# Autodesk Inventor assembly: Gripper Assembly
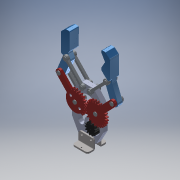
[picture p0: Inventor's stored thumbnail of the model, 180x180]
Saved by Autodesk Inventor 2019 (Build 230136000, 136)
## iProperties
Created: 2020-11-14
Part Number: Gripper Assembly
Document SubType Name: Assembly
Designer: micha
Author: micha
## Documents named in this file (12)
- D:\Files\ASU - Faculty of Engineering\Semester 10 - Spring 2021\Industrial Mechanisms and Robotics - MCT331\Four Bar Gripper Project\Gripper Assembly.iam
- D:\Files\ASU - Faculty of Engineering\Semester 10 - Spring 2021\Industrial Mechanisms and Robotics - MCT331\Four Bar Gripper Project\Part3_Base Gripper.ipt
- D:\Files\ASU - Faculty of Engineering\Semester 10 - Spring 2021\Industrial Mechanisms and Robotics - MCT331\Four Bar Gripper Project\Part4_Penggerak Kanan.ipt
- D:\Files\ASU - Faculty of Engineering\Semester 10 - Spring 2021\Industrial Mechanisms and Robotics - MCT331\Four Bar Gripper Project\Part5_Penggerak Kiri.ipt
- D:\Files\ASU - Faculty of Engineering\Semester 10 - Spring 2021\Industrial Mechanisms and Robotics - MCT331\Four Bar Gripper Project\Part1_Penjepit.ipt
- D:\Files\ASU - Faculty of Engineering\Semester 10 - Spring 2021\Industrial Mechanisms and Robotics - MCT331\Four Bar Gripper Project\Part2_Penyangga.ipt
- D:\Files\ASU - Faculty of Engineering\Semester 10 - Spring 2021\Industrial Mechanisms and Robotics - MCT331\Four Bar Gripper Project\Part6_Penyambung.ipt
- D:\Files\ASU - Faculty of Engineering\Semester 10 - Spring 2021\Industrial Mechanisms and Robotics - MCT331\Four Bar Gripper Project\Part7_Gripper to arm.ipt
- D:\Files\ASU - Faculty of Engineering\Semester 10 - Spring 2021\Industrial Mechanisms and Robotics - MCT331\Four Bar Gripper Project\Part8_to servo.ipt
- D:\Files\ASU - Faculty of Engineering\Semester 10 - Spring 2021\Industrial Mechanisms and Robotics - MCT331\Four Bar Gripper Project\Part1_Penjepit_V.ipt
- D:\Files\ASU - Faculty of Engineering\Semester 10 - Spring 2021\Industrial Mechanisms and Robotics - MCT331\Four Bar Gripper Project\Part1_Penjepit_Cutted.ipt
- D:\Files\ASU - Faculty of Engineering\Semester 10 - Spring 2021\Industrial Mechanisms and Robotics - MCT331\Four Bar Gripper Project\Part1_Penjepit_V_Cutted.ipt
## Components (29 placed, 10 different names)
1. Part3_Base Gripper:1
2. Part4_Penggerak Kanan:1
3. Part5_Penggerak Kiri:1
4. Part1_Penjepit:2 — Flush:1, Mate:3, Flush:2
5. Part2_Penyangga:1
6. Part2_Penyangga:2
7. Part1_Penjepit:6 — Mate:5
8. Part3_Base Gripper:2
9. Part1_Penjepit:7 — Flush:5, Flush:6, Mate:6, Flush:7, Flush:8
10. Part1_Penjepit:8 — Mate:4, Flush:3, Flush:4
11. Part2_Penyangga:4
12. Part2_Penyangga:5
13. Part2_Penyangga:6
14. Part2_Penyangga:7
15. Part6_Penyambung:1
16. Part7_Gripper to arm:1
17. Part6_Penyambung:2
18. Part6_Penyambung:4
19. Part6_Penyambung:6
20. Part6_Penyambung:8
21. Part6_Penyambung:10
22. Part6_Penyambung:12
23. Part6_Penyambung:14
24. Part7_Gripper to arm:2
25. Part8_to servo:2
26. Part1_Penjepit_Cutted:1 — Flush:1, Mate:3, Flush:2
27. Part1_Penjepit_Cutted:2 — Mate:4, Flush:3, Flush:4
28. Part1_Penjepit_V_Cutted:1 — Mate:5, Flush:5, Flush:6
29. Part1_Penjepit_V_Cutted:2 — Mate:6, Flush:7, Flush:8
## Relationships (12: Flush 8, Mate 4)
- Flush:1: Part1_Penjepit:2 ↔ Part1_Penjepit_Cutted:1
- Mate:3: Part1_Penjepit:2 ↔ Part1_Penjepit_Cutted:1
- Flush:2: Part1_Penjepit:2 ↔ Part1_Penjepit_Cutted:1
- Mate:4: Part1_Penjepit:8 ↔ Part1_Penjepit_Cutted:2
- Flush:3: Part1_Penjepit:8 ↔ Part1_Penjepit_Cutted:2
- Flush:4: Part1_Penjepit:8 ↔ Part1_Penjepit_Cutted:2
- Mate:5: Part1_Penjepit:6 ↔ Part1_Penjepit_V_Cutted:1
- Flush:5: Part1_Penjepit:7 ↔ Part1_Penjepit_V_Cutted:1
- Flush:6: Part1_Penjepit:7 ↔ Part1_Penjepit_V_Cutted:1
- Mate:6: Part1_Penjepit:7 ↔ Part1_Penjepit_V_Cutted:2
- Flush:7: Part1_Penjepit:7 ↔ Part1_Penjepit_V_Cutted:2
- Flush:8: Part1_Penjepit:7 ↔ Part1_Penjepit_V_Cutted:2
